# Autodesk Inventor assembly: Band assembly
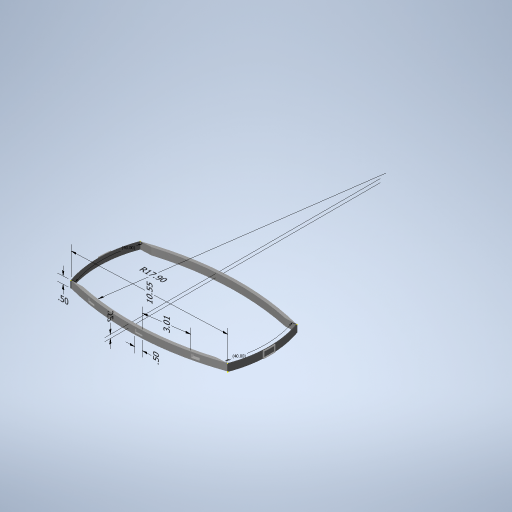
[picture p0: Inventor's stored thumbnail of the model, 512x512]
Saved by Autodesk Inventor 2024 (Build 280153000, 153)
## iProperties
Created: 2025-11-15
Part Number: Band assembly
Document SubType Name: Assembly
Designer: garys
Author: garys
## Documents named in this file (4)
- \\nas01.itap.purdue.edu\puhome\My Documents\senior design\Band assembly.iam
- \\nas01.itap.purdue.edu\puhome\My Documents\senior design\front_back band.ipt
- \\nas01.itap.purdue.edu\puhome\My Documents\senior design\side band.ipt
- \\nas01.itap.purdue.edu\puhome\My Documents\senior design\buckle.ipt
## Components (6 placed, 3 different names)
1. front_back band:1 — Mate:1, Mate:4, Flush:2
2. front_back band:2 — Mate:2, Mate:3, Flush:1, Flush:3
3. side band:1 — Mate:1, Mate:2, Flush:1, Flush:2, Mate:5, Flush:4
4. side band:2 — Mate:3, Mate:4, Flush:3, Mate:6, Flush:5
5. buckle:1 — Mate:5, Flush:4
6. buckle:2 — Mate:6, Flush:5
## Relationships (11: Mate 6, Flush 5)
- Mate:1: front_back band:1 ↔ side band:1
- Mate:2: front_back band:2 ↔ side band:1
- Mate:3: front_back band:2 ↔ side band:2
- Mate:4: front_back band:1 ↔ side band:2
- Flush:1: front_back band:2 ↔ side band:1
- Flush:2: front_back band:1 ↔ side band:1
- Flush:3: front_back band:2 ↔ side band:2
- Mate:5 (1.27 mm): side band:1 ↔ buckle:1
- Flush:4: side band:1 ↔ buckle:1
- Mate:6 (1.27 mm): side band:2 ↔ buckle:2
- Flush:5: side band:2 ↔ buckle:2
